# Autodesk Inventor assembly: general
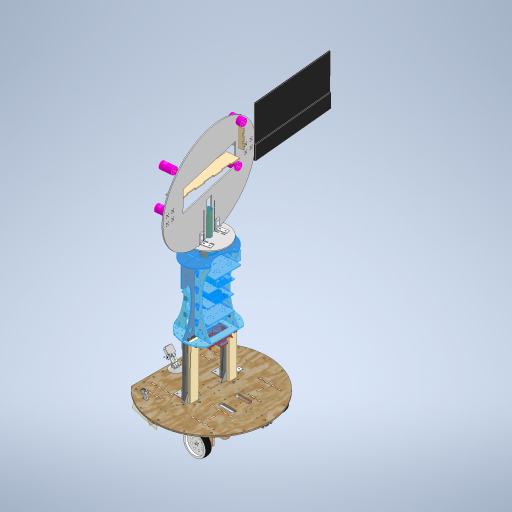
[picture p0: Inventor's stored thumbnail of the model, 512x512]
Saved by Autodesk Inventor 2023 (Build 270158000, 158)
## iProperties
Created: 2024-12-19
Part Number: general
Document SubType Name: Assembly
Designer: DELL
Author: DELL
## Documents named in this file (5)
- \\sch239.net\UserHomes\Students\other\baranovaem\cheburashka\Cheburashka-main\Cheburashka_construction\general.iam
- \\sch239.net\UserHomes\Students\other\baranovaem\cheburashka\Cheburashka-main\Cheburashka_construction\platform\platform.iam
- \\sch239.net\UserHomes\Students\other\baranovaem\cheburashka\Cheburashka-main\Cheburashka_construction\korpus\korp.iam
- \\sch239.net\UserHomes\Students\other\baranovaem\cheburashka\Cheburashka-main\Cheburashka_construction\platform\8bc17c1464c21f56fb2a3979b7c6b729.ipt
- D:\лицо\Сборка1.iam
## Components (7 placed, 4 different names)
1. platform:1 [sub-assembly] — Заподлицо:1, Совмещение:4, Совмещение:5, Совмещение:7, Совмещение:8, Совмещение:10, Совмещение:11, Совмещение:13, Совмещение:14
2. korp:1 [sub-assembly] — Заподлицо:1, Совмещение:3, Совмещение:6, Совмещение:9, Совмещение:12, Совмещение:15, Касательность:1, Совмещение:16, Совмещение:17
3. 8bc17c1464c21f56fb2a3979b7c6b729:1 — Совмещение:3, Совмещение:4, Совмещение:5
4. 8bc17c1464c21f56fb2a3979b7c6b729:2 — Совмещение:6, Совмещение:7, Совмещение:8
5. 8bc17c1464c21f56fb2a3979b7c6b729:3 — Совмещение:9, Совмещение:10, Совмещение:11
6. 8bc17c1464c21f56fb2a3979b7c6b729:4 — Совмещение:12, Совмещение:13, Совмещение:14
7. Сборка1:1 [sub-assembly] — Совмещение:15, Касательность:1, Совмещение:16, Совмещение:17
## Relationships (17: Mate 15, Flush 1, Tangent 1)
- Заподлицо:1 [Flush]: platform:1 ↔ korp:1
- Совмещение:3 [Mate]: korp:1 ↔ 8bc17c1464c21f56fb2a3979b7c6b729:1
- Совмещение:4 [Mate]: platform:1 ↔ 8bc17c1464c21f56fb2a3979b7c6b729:1
- Совмещение:5 [Mate]: platform:1 ↔ 8bc17c1464c21f56fb2a3979b7c6b729:1
- Совмещение:6 [Mate]: korp:1 ↔ 8bc17c1464c21f56fb2a3979b7c6b729:2
- Совмещение:7 [Mate]: platform:1 ↔ 8bc17c1464c21f56fb2a3979b7c6b729:2
- Совмещение:8 [Mate]: platform:1 ↔ 8bc17c1464c21f56fb2a3979b7c6b729:2
- Совмещение:9 [Mate]: korp:1 ↔ 8bc17c1464c21f56fb2a3979b7c6b729:3
- Совмещение:10 [Mate]: platform:1 ↔ 8bc17c1464c21f56fb2a3979b7c6b729:3
- Совмещение:11 [Mate]: platform:1 ↔ 8bc17c1464c21f56fb2a3979b7c6b729:3
- Совмещение:12 [Mate]: korp:1 ↔ 8bc17c1464c21f56fb2a3979b7c6b729:4
- Совмещение:13 [Mate]: platform:1 ↔ 8bc17c1464c21f56fb2a3979b7c6b729:4
- Совмещение:14 [Mate]: platform:1 ↔ 8bc17c1464c21f56fb2a3979b7c6b729:4
- Совмещение:15 [Mate]: korp:1 ↔ Сборка1:1
- Касательность:1 [Tangent]: korp:1 ↔ Сборка1:1
- Совмещение:16 [Mate]: korp:1 ↔ Сборка1:1
- Совмещение:17 [Mate]: korp:1 ↔ Сборка1:1
